# Autodesk Inventor assembly: Plates
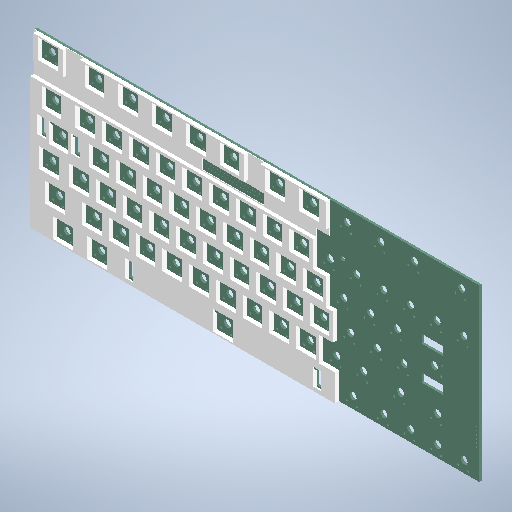
[picture p0: Inventor's stored thumbnail of the model, 512x512]
Saved by Autodesk Inventor 2025 (Build 290162000, 162)
## iProperties
Created: 2024-08-01
Part Number: Plates
Document SubType Name: Assembly
Designer: adam
Author: adam
## iProperties of the stored document _autosave-A600KBv2_PCB.ipt
Created: 2024-08-01
Part Number: _autosave-A600KBv2_PCB
Material: Generic
Document SubType Name: Modeling
Designer: adam
Density: 1 g/cm^3
Appearance: Default
Author: adam
## iProperties of the stored document A600KBv2.iam
Created: 2024-08-01
Part Number: A600KBv2 1
Description: KiCad electronic assembly
Document SubType Name: Assembly
Designer: adam
Authority: Unknown
Company: Kicad
Title: A600KBv2.step
Author: Pcbnew
Sending System: KiCad to STEP converter
Preprocessor: Open CASCADE STEP processor 7.8
## Documents named in this file (5)
- **C:\Users\adam\Projects\A600KBv2\3dprint\Keyboard Plates\Plates.iam*LocalDocs*xAaaaqtaaAaaaaaaaAaaaaeg12a*_autosave-A600KBv2_PCB.ipt
- **C:\Users\adam\Projects\A600KBv2\3dprint\Keyboard Plates\Plates.iam*LocalDocs*xAaaaafcaAaaaaaaaAaaaq0x1Jf*A600KBv2.iam
- C:\Users\adam\Projects\A600KBv2\3dprint\Keyboard Plates\Plates.iam
- C:\Users\adam\Projects\SEE222\Pet Food Dispenser\3dprint\Left plate.ipt
- C:\Users\adam\Projects\A600KBv2\3dprint\Keyboard Plates\A600KBv2.step
## Components (2 placed, 2 different names)
1. A600KBv2:1 [sub-assembly] — Flush:1
2. Left plate:1 — Flush:1
## Relationships (1: Flush 1)
- Flush:1: A600KBv2:1 ↔ Left plate:1
